# Autodesk Inventor assembly: Pully 34mmx10mm
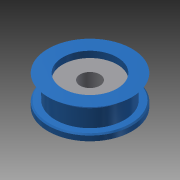
[picture p0: Inventor's stored thumbnail of the model, 180x180]
Saved by Autodesk Inventor 2013 (Build 170138000, 138)
## iProperties
Created: 2017-01-25
Part Number: Pully 34mmx10mm
Document SubType Name: Assembly
Designer: Herman de Vries
Author: Herman de Vries
## Documents named in this file (3)
- D:\Projects\Inventor\PaintBoid\Pully 34mmx12mm.iam
- D:\Projects\Inventor\PaintBoid\bearing 8mmx22mmx7mm.ipt
- D:\Projects\Inventor\PaintBoid\pully 22mmx34mmx12mm.ipt
## Components (2 placed, 2 different names)
1. bearing 8mmx22mmx7mm:1 — Insert:1
2. pully 22mmx34mmx12mm:1 — Insert:1
## Relationships (1: Insert 1)
- Insert:1 (-2.5 mm): bearing 8mmx22mmx7mm:1 ↔ pully 22mmx34mmx12mm:1
